# Autodesk Inventor assembly: Assembly5
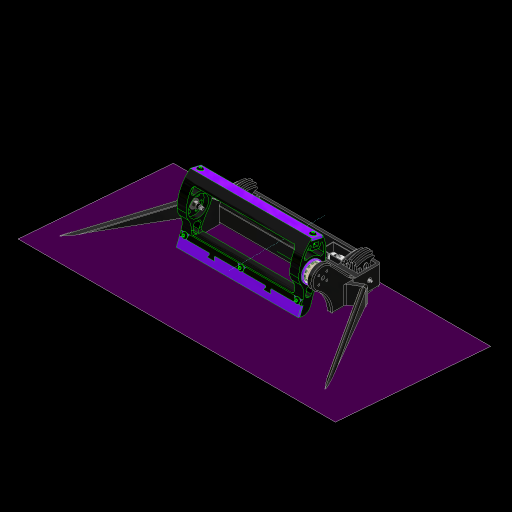
[picture p0: Inventor's stored thumbnail of the model, 512x512]
Saved by Autodesk Inventor 2023 (Build 270158000, 158)
## iProperties
Created: 2023-02-15
Part Number: Assembly5
Document SubType Name: Assembly
Designer: tandu
Mass: 512.824 g
Surface Area: 1841.01 cm^2
Volume: 285.129 cm^3
Density: 1.79857 g/cm^3
Author: tandu
## Documents named in this file (12)
- C:\Users\tandu\Documents\GrabCAD\Insomnia 2020\Versions\10 Shuffler\ShufflerVersion\SVAssembly5.iam
- C:\Users\tandu\Documents\GrabCAD\Insomnia 2020\Versions\10 Shuffler\ShufflerVersion\Weapon\DrumAssembly.iam
- C:\Users\tandu\Documents\GrabCAD\Insomnia 2020\Versions\10 Shuffler\ShufflerVersion\BatteryMockup.ipt
- C:\Users\tandu\Documents\GrabCAD\Insomnia 2020\Versions\9 Comically Large Weapon 9 28 22\2207 5 fixed motor.ipt
- C:\Users\tandu\Documents\GrabCAD\Insomnia 2020\Versions\10 Shuffler\ShufflerVersion\WedgeTPUPiece.ipt
- C:\Users\tandu\Documents\GrabCAD\Insomnia 2020\Versions\10 Shuffler\ShufflerVersion\WedgeTPUPiece_MIR.ipt
- C:\Users\tandu\Documents\GrabCAD\Insomnia 2020\Versions\10 Shuffler\ShufflerVersion\90417A126_Phillips Rounded Head Thread-Forming Screws.ipt
- C:\Users\tandu\Documents\GrabCAD\Insomnia 2020\Versions\9 Comically Large Weapon 9 28 22\57155K571_Flanged Ball Bearing.ipt
- C:\Users\tandu\Documents\GrabCAD\Insomnia 2020\Versions\10 Shuffler\WheeledVersion\94361A593_Short-Thread Alloy Steel Shoulder Screw.ipt
- C:\Users\tandu\Documents\GrabCAD\Insomnia 2020\Versions\10 Shuffler\ShufflerVersion\Weapon\90237A110_High-Strength Steel Nylon-Insert Locknuts.ipt
- C:\Users\tandu\Documents\GrabCAD\Insomnia 2020\Versions\10 Shuffler\ShufflerVersion\ChassisShuffler.ipt
- C:\Users\tandu\Documents\GrabCAD\Insomnia 2020\Versions\10 Shuffler\ShufflerVersion\Shuffler\Shuffler.iam
## Components (22 placed, 11 different names)
1. ChassisShuffler:1 — Insert:21, Insert:22
2. BatteryMockup:1
3. WedgeTPUPiece:1 — Mate:5
4. WedgePiece_MIR:1 — Mate:6
5. Shuffler:1 [sub-assembly] — Insert:21
6. Shuffler:2 [sub-assembly] — Insert:22
7. 90417A126_Phillips Rounded Head Thread-Forming Screws:5
8. 90417A126_Phillips Rounded Head Thread-Forming Screws:6
9. 90417A126_Phillips Rounded Head Thread-Forming Screws:7
10. 90417A126_Phillips Rounded Head Thread-Forming Screws:8
11. 90417A126_Phillips Rounded Head Thread-Forming Screws:9
12. 90417A126_Phillips Rounded Head Thread-Forming Screws:10
13. 90417A126_Phillips Rounded Head Thread-Forming Screws:1
14. 90417A126_Phillips Rounded Head Thread-Forming Screws:2
15. 90417A126_Phillips Rounded Head Thread-Forming Screws:3
16. 90417A126_Phillips Rounded Head Thread-Forming Screws:4
17. DrumAssembly:1 [sub-assembly] — Insert:5, Insert:17, Insert:18
18. 2207 5 fixed motor:1 — Insert:5
19. 57155K571_Flanged Ball Bearing:2 — Insert:17
20. 57155K571_Flanged Ball Bearing:3 — Insert:18, Insert:20
21. 94361A593_Short-Thread Alloy Steel Shoulder Screw:1
22. 90237A110_High-Strength Steel Nylon-Insert Locknuts:1 — Insert:20
## Relationships (24: Insert 17, Mate 7)
- [Mate]: ChassisShuffler:1 ↔ BatteryMockup:1
- [Mate]: ChassisShuffler:1 ↔ BatteryMockup:1
- [Insert]: ChassisShuffler:1 ↔ 2207 5 fixed motor:1
- [Insert]: ChassisShuffler:1 ↔ 2207 5 fixed motor:1
- Insert:5: DrumAssembly:1 ↔ 2207 5 fixed motor:1
- [Mate]: ChassisShuffler:1 ↔ WedgeTPUPiece:1
- [Mate]: ChassisShuffler:1 ↔ WedgePiece_MIR:1
- [Insert]: ChassisShuffler:1 ↔ WedgeTPUPiece:1
- [Insert]: ChassisShuffler:1 ↔ WedgeTPUPiece:1
- [Insert]: ChassisShuffler:1 ↔ WedgePiece_MIR:1
- [Insert]: ChassisShuffler:1 ↔ WedgePiece_MIR:1
- [Insert]: ChassisShuffler:1 ↔ 90417A126_Phillips Rounded Head Thread-Forming Screws:3
- [Insert]: ChassisShuffler:1 ↔ 90417A126_Phillips Rounded Head Thread-Forming Screws:1
- [Insert]: ChassisShuffler:1 ↔ 90417A126_Phillips Rounded Head Thread-Forming Screws:2
- [Insert]: ChassisShuffler:1 ↔ 90417A126_Phillips Rounded Head Thread-Forming Screws:4
- Insert:17: DrumAssembly:1 ↔ 57155K571_Flanged Ball Bearing:2
- Insert:18: DrumAssembly:1 ↔ 57155K571_Flanged Ball Bearing:3
- [Insert]: ChassisShuffler:1 ↔ 94361A593_Short-Thread Alloy Steel Shoulder Screw:1
- Insert:20: 57155K571_Flanged Ball Bearing:3 ↔ 90237A110_High-Strength Steel Nylon-Insert Locknuts:1
- Mate:5: WedgeTPUPiece:1
- Mate:6: WedgePiece_MIR:1
- Mate:7
- Insert:21: ChassisShuffler:1 ↔ Shuffler:1
- Insert:22: ChassisShuffler:1 ↔ Shuffler:2
